# Autodesk Inventor assembly: TBCK-MA5150
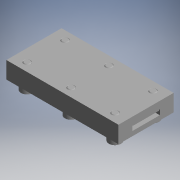
[picture p0: Inventor's stored thumbnail of the model, 180x180]
Saved by Autodesk Inventor 2017.3 (Build 213256000, 256)
## iProperties
Category: PARTsolutions
Company: MISUMI
Part Number: TBCK-MA5150
Catalog Web Link: www.cadenas.de
Description: TBCK_XL, TBCK_L, TBCK_H, TBCK_S3M, TBCK_S5M, TBCK_S8M, TBCK_MA3, TBCK_MA5, TBCK_MA8, TBCK_T5, TBCK_T10, TBCK_AT5, TBCK_AT10-Metal Fittings for Timing Belts - Press Prevention Type
Vendor: MISUMI
Document SubType Name: Assembly
Designer: partserver
Manufacturer: MISUMI
Mass: 19.0024 g
Surface Area: 134.092 cm^2
Volume: 19.0024 cm^3
Density: 1 g/cm^3
Title: TBCK-MA5150
Author: Cadenas PARTsolutions
Comments: Metal Fittings for Timing Belts - Press Prevention Type
PSOL_IDENT_0: {$CADENAS_DATA\23d-libs\misumi\metric\48_timing_belts\tbck_asmtab.prj},288 {VTYP=3D},{STYP=ASSTAB},{
PSOL_IDENT_1: NB=TBCK-MA5150},{LINA=TBCK-MA5150},{NN=TBCK_XL, TBCK_L, TBCK_H, TBCK_S3M, TBCK_S5M, TBCK_S8M, TBCK_M
PSOL_IDENT_2: A3, TBCK_MA5, TBCK_MA8, TBCK_T5, TBCK_T10, TBCK_AT5, TBCK_AT10},{DATE=30.06.2021 13:24:11},{GEOMDATE=
PSOL_IDENT_3: 11.02.2010},{VERSION=},{LINEID=120},{WBVAR=BNW},{WBNUMERIC=}  {NB=TBCK-MA5150},{LINA=TBCK-MA5150},{K
PSOL_IDENT_4: T=DUMMY},{PN=TBCK-MA5150},{TYPE=TBCK},{MAT=A6N01-T5},{ST=Clear Anodizing},{AC=Hexagon Socket Head Ca
PSOL_IDENT_5: p Screw},{TB=MA5},{BNW=150},{BNW1='100','100','150','150','250','250'},{W=15.0},{A=65},{B=32},{T1=6}
PSOL_IDENT_6: ,{T2=5.5},{T3=2.90},{HH=1.70},{L=51},{P=22},{M=M4},{M1=4},{DD=4.5},{AB=M4-10},{AB1=10},{NMH=6},{PPAT
PSOL_IDENT_7: H=tbck_rack_asmtpl.prj}
NB: TBCK-MA5150
NN: TBCK_XL, TBCK_L, TBCK_H, TBCK_S3M, TBCK_S5M, TBCK_S8M, TBCK_MA3, TBCK_MA5, TBCK_MA8, TBCK_T5, TBCK_T10, TBCK_AT5, TBCK_AT10
NT: Metal Fittings for Timing Belts - Press Prevention Type
NBSYN: $PN.
LINA: TBCK-MA5150
CATALOG: Misumi
PN: TBCK-MA5150
MAT: A6N01-T5
ST: Clear Anodizing
AC: Hexagon Socket Head Cap Screw
TB: MA5
BNW: 150
W: 15
A: 65
B: 32
T1: 6
T2: 5.5
T3: 2.9
HH: 1.7
L: 51
P: 22
M: M4
DD: 4.5
AB: M4-10
NMH: 6
SUPPLIER: MISUMI
ARTICLENO: TBCK-MA5150
BOMINFO: TBCK-MA5150
CREATOR: CADENAS GmbH
## Documents named in this file (4)
- e:\temp\worker_15\temp\exporttempdir_932_62_xUOI9\format_0\TBCK-MA5150.iam
- e:\temp\worker_15\temp\exporttempdir_932_62_xUOI9\format_0\TBCKsupport_plate-MA5150_r.ipt
- e:\temp\worker_15\temp\exporttempdir_932_62_xUOI9\format_0\TBCKsupport_plate-MA5150_support_plate.ipt
- e:\temp\worker_15\temp\exporttempdir_932_62_xUOI9\format_0\CB4-10_1.ipt
## Components (8 placed, 3 different names)
1. TBCKsupport_plate-MA5150_r:1 — tbck_XY@1 <-> tbck_XY@2, tbck_Z@1 <-> tbck_Z@2, tbck_YZ@1 <-> tbck_YZ@2
2. TBCKsupport_plate-MA5150_support_plate:1 — tbck_XY@1 <-> tbck_XY@2, tbck_Z@1 <-> tbck_Z@2, tbck_YZ@1 <-> tbck_YZ@2, tbck_holes_1_Z@2 <-> screw1_Z@3, tbck_holes_2_Z@2 <-> screw1_Z@4, tbck_holes_3_Z@2 <-> screw1_Z@5, tbck_hole_1_Z@2 <-> screw1_Z@6, tbck_hole_2_Z@2 <-> screw1_Z@7, tbck_hole_3_Z@2 <-> screw1_Z@8
3. CB4-10_1:1 — tbck_holes_1_Z@2 <-> screw1_Z@3
4. CB4-10_1:2 — tbck_holes_2_Z@2 <-> screw1_Z@4
5. CB4-10_1:3 — tbck_holes_3_Z@2 <-> screw1_Z@5
6. CB4-10_1:4 — tbck_hole_1_Z@2 <-> screw1_Z@6
7. CB4-10_1:5 — tbck_hole_2_Z@2 <-> screw1_Z@7
8. CB4-10_1:6 — tbck_hole_3_Z@2 <-> screw1_Z@8
## Relationships (9: Mate 8, Angle 1)
- tbck_XY@1 <-> tbck_XY@2 [Mate]: TBCKsupport_plate-MA5150_r:1 ↔ TBCKsupport_plate-MA5150_support_plate:1
- tbck_Z@1 <-> tbck_Z@2 [Mate]: TBCKsupport_plate-MA5150_r:1 ↔ TBCKsupport_plate-MA5150_support_plate:1
- tbck_YZ@1 <-> tbck_YZ@2 [Angle] (0 deg): TBCKsupport_plate-MA5150_r:1 ↔ TBCKsupport_plate-MA5150_support_plate:1
- tbck_holes_1_Z@2 <-> screw1_Z@3 [Mate]: TBCKsupport_plate-MA5150_support_plate:1 ↔ CB4-10_1:1
- tbck_holes_2_Z@2 <-> screw1_Z@4 [Mate]: TBCKsupport_plate-MA5150_support_plate:1 ↔ CB4-10_1:2
- tbck_holes_3_Z@2 <-> screw1_Z@5 [Mate]: TBCKsupport_plate-MA5150_support_plate:1 ↔ CB4-10_1:3
- tbck_hole_1_Z@2 <-> screw1_Z@6 [Mate]: TBCKsupport_plate-MA5150_support_plate:1 ↔ CB4-10_1:4
- tbck_hole_2_Z@2 <-> screw1_Z@7 [Mate]: TBCKsupport_plate-MA5150_support_plate:1 ↔ CB4-10_1:5
- tbck_hole_3_Z@2 <-> screw1_Z@8 [Mate]: TBCKsupport_plate-MA5150_support_plate:1 ↔ CB4-10_1:6
